# Autodesk Inventor assembly: Assembly1st
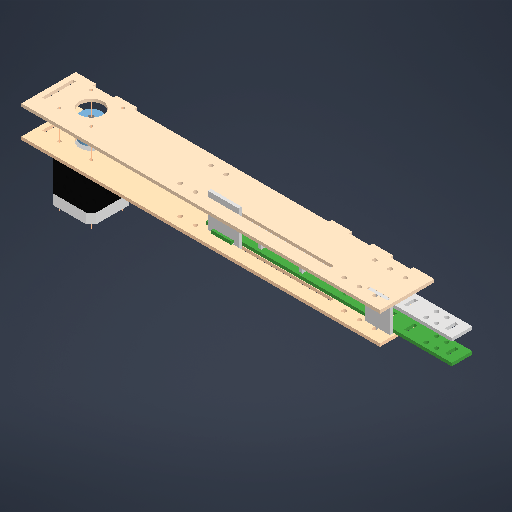
[picture p0: Inventor's stored thumbnail of the model, 512x512]
Saved by Autodesk Inventor 2027 (Build 310192000, 192)
## iProperties
Created: 2026-05-09
Part Number: Assembly1st
Document SubType Name: Assembly
Designer: alexy
Author: alexy
## Documents named in this file (10)
- C:\Users\alexy\OneDrive\文件\Carinventor\1stmodel\Assembly1st.iam
- C:\Users\alexy\OneDrive\文件\Carinventor\1stmodel\Nema 17 stepper motor.ipt
- C:\Users\alexy\OneDrive\文件\Carinventor\1stmodel\Sideboard.ipt
- C:\Users\alexy\OneDrive\文件\Carinventor\1stmodel\Backboard.ipt
- C:\Users\alexy\OneDrive\文件\Carinventor\1stmodel\Frontrail.ipt
- C:\Users\alexy\OneDrive\文件\Carinventor\1stmodel\Moving_rail.ipt
- C:\Users\alexy\OneDrive\文件\Carinventor\1stmodel\D_coupler.ipt
- C:\Users\alexy\OneDrive\文件\Carinventor\1stmodel\Middle_bar.ipt
- C:\Users\alexy\OneDrive\文件\Carinventor\1stmodel\Spring_holder.ipt
- C:\Users\alexy\OneDrive\文件\Carinventor\1stmodel\Spring_holder2.ipt
## Components (11 placed, 9 different names)
1. Nema 17 stepper motor:1 — Insert:1, Insert:2, Angle:1
2. Sideboard:1 — Insert:1, Flush:1, Flush:2, Mate:1, Mate:2, Mate:3, Mate:5, Mate:6, Mate:7, Mate:8, Mate:15, Mate:16
3. Sideboard:2 — Flush:1, Flush:2, Mate:4
4. Backboard:1 — Mate:1, Mate:2, Mate:3, Mate:4
5. Frontrail:1 — Mate:5, Mate:6, Mate:7
6. Moving_rail:1 — Mate:8, Mate:9, Mate:10, Mate:11, Mate:12, Mate:13, Mate:14, Mate:16
7. D_coupler:1 — Insert:2, Angle:1
8. Middle_bar:1 — Mate:9, Mate:10, Mate:11, Mate:15, Mate:17, Mate:18, Mate:19, Mate:20, Mate:21, Mate:22
9. Middle_bar:2 — Mate:12, Mate:13, Mate:14
10. Spring_holder:1 — Mate:17, Mate:18, Mate:19
11. Spring_holder2:1 — Mate:20, Mate:21, Mate:22
## Relationships (27: Mate 22, Insert 2, Flush 2, Angle 1)
- Insert:1: Nema 17 stepper motor:1 ↔ Sideboard:1
- Flush:1: Sideboard:1 ↔ Sideboard:2
- Flush:2: Sideboard:1 ↔ Sideboard:2
- Mate:1: Sideboard:1 ↔ Backboard:1
- Mate:2: Sideboard:1 ↔ Backboard:1
- Mate:3: Sideboard:1 ↔ Backboard:1
- Mate:4: Sideboard:2 ↔ Backboard:1
- Mate:5: Sideboard:1 ↔ Frontrail:1
- Mate:6: Sideboard:1 ↔ Frontrail:1
- Mate:7: Sideboard:1 ↔ Frontrail:1
- Mate:8: Sideboard:1 ↔ Moving_rail:1
- Insert:2 (4 mm): Nema 17 stepper motor:1 ↔ D_coupler:1
- Angle:1 (331 deg): Nema 17 stepper motor:1 ↔ D_coupler:1
- Mate:9: Moving_rail:1 ↔ Middle_bar:1
- Mate:10: Moving_rail:1 ↔ Middle_bar:1
- Mate:11: Moving_rail:1 ↔ Middle_bar:1
- Mate:12: Moving_rail:1 ↔ Middle_bar:2
- Mate:13: Moving_rail:1 ↔ Middle_bar:2
- Mate:14: Moving_rail:1 ↔ Middle_bar:2
- Mate:15 (0.5 mm): Sideboard:1 ↔ Middle_bar:1
- Mate:16: Sideboard:1 ↔ Moving_rail:1
- Mate:17: Middle_bar:1 ↔ Spring_holder:1
- Mate:18: Middle_bar:1 ↔ Spring_holder:1
- Mate:19: Middle_bar:1 ↔ Spring_holder:1
- Mate:20: Middle_bar:1 ↔ Spring_holder2:1
- Mate:21: Middle_bar:1 ↔ Spring_holder2:1
- Mate:22: Middle_bar:1 ↔ Spring_holder2:1
